# Autodesk Inventor assembly: Gearbox
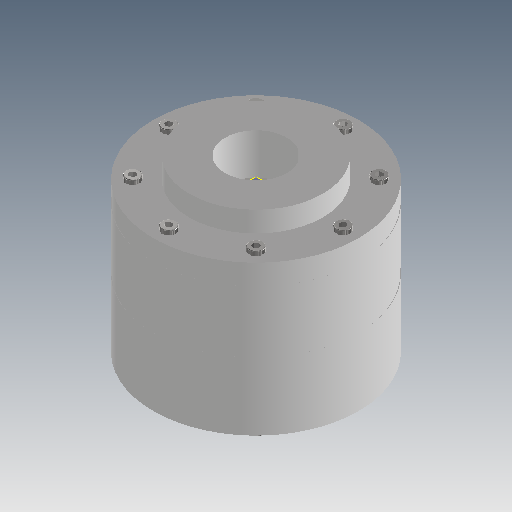
[picture p0: Inventor's stored thumbnail of the model, 512x512]
Saved by Autodesk Inventor 2020.3 (Build 243373010, 373A)
## iProperties
Created: 2021-05-01
Part Number: Gearbox
Document SubType Name: Assembly
Designer: marti
Author: marti
## Documents named in this file (10)
- C:\Users\marti\Documents\Inventor\RobotManipulateArm\17.4.2021 - Complete new IDEA\Gearbox.iam
- C:\Users\marti\Documents\Inventor\RobotManipulateArm\17.4.2021 - Complete new IDEA\Cycloidal gear 02.ipt
- C:\Users\marti\Documents\Inventor\RobotManipulateArm\17.4.2021 - Complete new IDEA\Cycloidal gear inner gear.ipt
- C:\Users\marti\Documents\Inventor\RobotManipulateArm\17.4.2021 - Complete new IDEA\Gearbox\Design Accelerator\Bearing1.iam
- C:\Users\marti\Documents\Inventor\RobotManipulateArm\17.4.2021 - Complete new IDEA\Cover of gearbox.ipt
- C:\Users\marti\Documents\Inventor\RobotManipulateArm\17.4.2021 - Complete new IDEA\Cycloidal gear cover front.ipt
- C:\Users\marti\Documents\Inventor\RobotManipulateArm\17.4.2021 - Complete new IDEA\Connection disc of gear.ipt
- C:\Users\marti\Documents\Inventor\RobotManipulateArm\17.4.2021 - Complete new IDEA\Cover of gearbox 2.ipt
- C:\Users\marti\Documents\Inventor\Content Center Files\R2020\en-US\ISO 4762(1)\DIN EN ISO 4762 - M4 x 16.ipt
- C:\Users\marti\Documents\Inventor\Content Center Files\R2020\en-US\ISO 4762(1)\DIN EN ISO 4762 - M4 x 40.ipt
## Components (25 placed, 9 different names)
1. Cycloidal gear inner gear:1 — Mate:1, Mate:2, Mate:3, Mate:4, Flush:1, Flush:2, Mate:13, Mate:14, Mate:21, Mate:27, Mate:28, Mate:31
2. Cycloidal gear 02:3 — Mate:5, Flush:2, Mate:6, Mate:8, Flush:4, Mate:24, Mate:25, Mate:26
3. Cycloidal gear 02:4 — Mate:3, Mate:4, Flush:1, Mate:5, Mate:6, Mate:7, Flush:3
4. Bearing:3 [sub-assembly] — Mate:7, Flush:3, Mate:16
5. Bearing:4 [sub-assembly] — Mate:8, Flush:4
6. Cover of gearbox:1 — Mate:13, Mate:14, Mate:16, Mate:34, Mate:35
7. Connection disc of gear:4 — Mate:24, Mate:25, Mate:26, Mate:29, Mate:30, Flush:5
8. Cycloidal gear cover front:2 — Mate:27, Mate:28, Mate:31, Mate:36, Mate:37
9. Cover of gearbox 2:2 — Mate:29, Mate:30, Flush:5
10. DIN EN ISO 4762 M4 x 16:2 — Mate:34, Mate:35
11. DIN EN ISO 4762 M4 x 16:3
12. DIN EN ISO 4762 M4 x 16:4
13. DIN EN ISO 4762 M4 x 16:5
14. DIN EN ISO 4762 M4 x 16:6
15. DIN EN ISO 4762 M4 x 16:7
16. DIN EN ISO 4762 M4 x 16:8
17. DIN EN ISO 4762 M4 x 16:9
18. DIN EN ISO 4762 M4 x 40:1 — Mate:36, Mate:37
19. DIN EN ISO 4762 M4 x 40:2
20. DIN EN ISO 4762 M4 x 40:3
21. DIN EN ISO 4762 M4 x 40:4
22. DIN EN ISO 4762 M4 x 40:5
23. DIN EN ISO 4762 M4 x 40:6
24. DIN EN ISO 4762 M4 x 40:7
25. DIN EN ISO 4762 M4 x 40:8
## Component patterns: (8 elements, first: DIN EN ISO 4762 M4 x 16:2), (8 elements, first: DIN EN ISO 4762 M4 x 40:1)
## Relationships (29: Mate 24, Flush 5)
- Mate:1: Cycloidal gear inner gear:1
- Mate:2: Cycloidal gear inner gear:1
- Mate:3: Cycloidal gear inner gear:1 ↔ Cycloidal gear 02:4
- Mate:4: Cycloidal gear inner gear:1 ↔ Cycloidal gear 02:4
- Flush:1: Cycloidal gear inner gear:1 ↔ Cycloidal gear 02:4
- Mate:5: Cycloidal gear 02:3 ↔ Cycloidal gear 02:4
- Flush:2: Cycloidal gear inner gear:1 ↔ Cycloidal gear 02:3
- Mate:6: Cycloidal gear 02:3 ↔ Cycloidal gear 02:4
- Mate:7: Cycloidal gear 02:4 ↔ Bearing:3
- Flush:3: Cycloidal gear 02:4 ↔ Bearing:3
- Mate:8: Cycloidal gear 02:3 ↔ Bearing:4
- Flush:4: Cycloidal gear 02:3 ↔ Bearing:4
- Mate:13: Cycloidal gear inner gear:1 ↔ Cover of gearbox:1
- Mate:14: Cycloidal gear inner gear:1 ↔ Cover of gearbox:1
- Mate:16: Bearing:3 ↔ Cover of gearbox:1
- Mate:21: Cycloidal gear inner gear:1
- Mate:24: Cycloidal gear 02:3 ↔ Connection disc of gear:4
- Mate:25: Cycloidal gear 02:3 ↔ Connection disc of gear:4
- Mate:26: Cycloidal gear 02:3 ↔ Connection disc of gear:4
- Mate:27: Cycloidal gear inner gear:1 ↔ Cycloidal gear cover front:2
- Mate:28: Cycloidal gear inner gear:1 ↔ Cycloidal gear cover front:2
- Mate:29: Connection disc of gear:4 ↔ Cover of gearbox 2:2
- Mate:30: Connection disc of gear:4 ↔ Cover of gearbox 2:2
- Flush:5: Connection disc of gear:4 ↔ Cover of gearbox 2:2
- Mate:31: Cycloidal gear inner gear:1 ↔ Cycloidal gear cover front:2
- Mate:34: Cover of gearbox:1 ↔ DIN EN ISO 4762 M4 x 16:2
- Mate:35: Cover of gearbox:1 ↔ DIN EN ISO 4762 M4 x 16:2
- Mate:36: Cycloidal gear cover front:2 ↔ DIN EN ISO 4762 M4 x 40:1
- Mate:37: Cycloidal gear cover front:2 ↔ DIN EN ISO 4762 M4 x 40:1
